# Autodesk Inventor assembly: Rama_oparcia
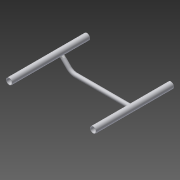
[picture p0: Inventor's stored thumbnail of the model, 180x180]
Saved by Autodesk Inventor 2015 (Build 190159000, 159)
## iProperties
Created: 2015-11-22
Part Number: Rama_oparcia
Document SubType Name: Weldment
Designer: graaapsik
Weld Material: Aluminium AW-7020
Author: graaapsik
## Documents named in this file (3)
- C:\Users\EriveltonDell\Documents\Centro Universitário da FEI\Wheelchair\CADEIRA DE RODAS - DESENHO\Model\Rama_oparcia.iam
- C:\Users\EriveltonDell\Documents\Centro Universitário da FEI\Wheelchair\CADEIRA DE RODAS - DESENHO\Model\Rura_pozioma_oparcia.ipt
- C:\Users\EriveltonDell\Documents\Centro Universitário da FEI\Wheelchair\CADEIRA DE RODAS - DESENHO\Model\Rura_pionowa_oparcia.ipt
## Components (3 placed, 2 different names)
1. Rura_pozioma_oparcia:1 — Zestawiający:3, Zestawiający:4
2. Rura_pionowa_oparcia:1 — Zestawiający:1, Zestawiający:2, Zestawiający:3, Równoległy:1, Zestawiający:4
3. Rura_pionowa_oparcia:2 — Zestawiający:1, Zestawiający:2, Równoległy:1
## Relationships (5: Mate 4, Flush 1)
- Zestawiający:1 [Mate] (432 mm): Rura_pionowa_oparcia:1 ↔ Rura_pionowa_oparcia:2
- Zestawiający:2 [Mate]: Rura_pionowa_oparcia:1 ↔ Rura_pionowa_oparcia:2
- Zestawiający:3 [Mate] (16 mm): Rura_pozioma_oparcia:1 ↔ Rura_pionowa_oparcia:1
- Równoległy:1 [Flush]: Rura_pionowa_oparcia:1 ↔ Rura_pionowa_oparcia:2
- Zestawiający:4 [Mate] (134 mm): Rura_pozioma_oparcia:1 ↔ Rura_pionowa_oparcia:1
